# Autodesk Inventor assembly: assembly wheel
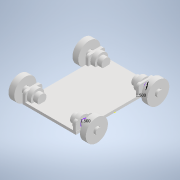
[picture p0: Inventor's stored thumbnail of the model, 180x180]
Saved by Autodesk Inventor 2021 (Build 250183000, 183)
## iProperties
Created: 2021-03-02
Part Number: assembly wheel
Document SubType Name: Assembly
Designer: K.V
Author: K.V
## Documents named in this file (4)
- C:\Users\K.V\OneDrive\Documents\assembly wheel.iam
- C:\Users\K.V\OneDrive\Documents\base final 1.ipt
- C:\Users\K.V\OneDrive\Documents\new wheel.ipt
- C:\Users\K.V\OneDrive\Documents\wheel final.ipt
## Components (9 placed, 3 different names)
1. base final 1:1 — Insert:1, Insert:3, Rigid:1, Rigid:2
2. new wheel:2 — Insert:1, Cylindrical:2
3. new wheel:4 — Insert:3, Cylindrical:3
4. new wheel:5 — Rigid:1, Rigid:3
5. new wheel:6 — Rigid:2, Cylindrical:1
6. wheel final:1 — Cylindrical:2
7. wheel final:2 — Cylindrical:1
8. wheel final:3 — Rigid:3
9. wheel final:4 — Cylindrical:3
## Relationships (8: WeldJoint 3, CylindricalJoint 3, Insert 2)
- Insert:1 (-76.2 mm): base final 1:1 ↔ new wheel:2
- Insert:3: base final 1:1 ↔ new wheel:4
- Rigid:1 [WeldJoint] (33.02 mm): base final 1:1 ↔ new wheel:5
- Rigid:2 [WeldJoint]: base final 1:1 ↔ new wheel:6
- Cylindrical:1: new wheel:6 ↔ wheel final:2
- Cylindrical:2: new wheel:2 ↔ wheel final:1
- Rigid:3 [WeldJoint]: new wheel:5 ↔ wheel final:3
- Cylindrical:3: new wheel:4 ↔ wheel final:4
